# Autodesk Inventor assembly: 足全体
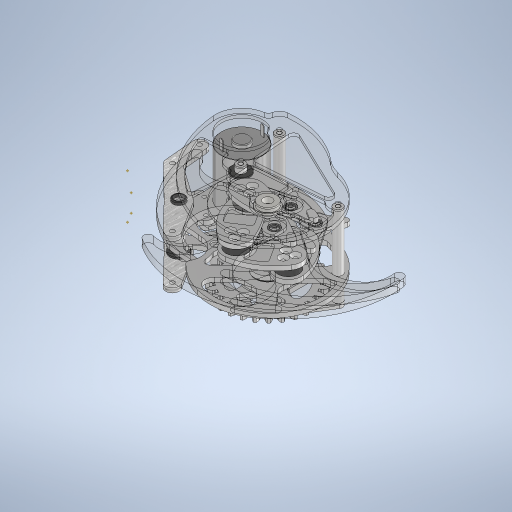
[picture p0: Inventor's stored thumbnail of the model, 512x512]
Saved by Autodesk Inventor 2023 (Build 270158000, 158)
## iProperties
Created: 2022-01-30
Part Number: 足全体
Document SubType Name: Assembly
Designer: acps
Author: acps
## Documents named in this file (6)
- C:\Users\acps\Documents\srdc\srdc_ksh\脚\足全体.iam
- C:\Users\acps\Documents\srdc\srdc_ksh\脚\アーノン.ipt
- C:\Users\acps\Documents\srdc\srdc_ksh\脚\足ユニット.iam
- C:\Users\acps\Documents\srdc\srdc_ksh\オイレス\w5f6-12a.ipt
- C:\Users\acps\Documents\srdc\srdc_ksh\スペーサ\l4.ipt
- C:\Users\acps\Documents\srdc\srdc_ksh\スペーサ\l19.ipt
## Components (8 placed, 5 different names)
1. 足ユニット:1 [sub-assembly] — Insert:8
2. アーノン:1 — Mate:6, Insert:3
3. アーノン:2 — Insert:10
4. w5f6-12a:1 — Mate:9, Insert:9, Insert:10
5. w5f6-12a:2 — Mate:6, Insert:3, Mate:10, Insert:6
6. l4:1 — Mate:10, Insert:6
7. l4:2 — Mate:9, Insert:9
8. l19:1 — Insert:8
## Relationships (8: Insert 5, Mate 3)
- Mate:6: アーノン:1 ↔ w5f6-12a:2
- Insert:3: アーノン:1 ↔ w5f6-12a:2
- Mate:9: w5f6-12a:1 ↔ l4:2
- Mate:10: w5f6-12a:2 ↔ l4:1
- Insert:6: w5f6-12a:2 ↔ l4:1
- Insert:8: 足ユニット:1 ↔ l19:1
- Insert:9: w5f6-12a:1 ↔ l4:2
- Insert:10: アーノン:2 ↔ w5f6-12a:1
